# Autodesk Inventor assembly: intake_base_MIR
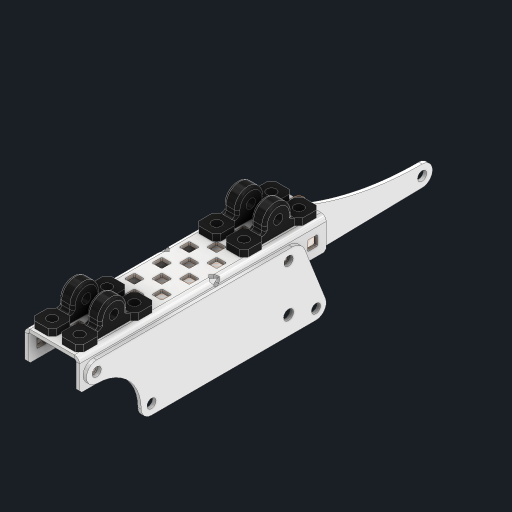
[picture p0: Inventor's stored thumbnail of the model, 512x512]
Saved by Autodesk Inventor 2024 (Build 280153000, 153)
## iProperties
Created: 2023-08-21
Part Number: intake_base_MIR
Document SubType Name: Assembly
Designer: Averey
Author: Averey
## Documents named in this file (5)
- D:\vex_robotics\hardware\cad\scrap_v0.1\intake\mirrored_parts\intake_base_MIR.iam
- D:\vex_robotics\hardware\cad\scrap_v0.1\intake\mirrored_parts\intake_base_MIR.ipt
- D:\vex_robotics\hardware\cad\scrap_v0.1\intake\mirrored_parts\intake_base_outer_MIR.ipt
- D:\vex_robotics\hardware\cad\scrap_v0.1\intake\mirrored_parts\LS Pillow Bearing Block_MIR.ipt
- D:\vex_robotics\hardware\cad\VEX-CAD-Inventor-1.41\Structure\C Channel\Aluminum 1x2x1\Alu C 1x2x1x9.ipt
## Components (7 placed, 4 different names)
1. intake_base_MIR:1 — Mate:7, Mate:8
2. intake_base_outer_MIR:1 — Insert:6, Mate:6
3. LS Pillow Bearing Block_MIR:1 — Insert:2, Mate:2
4. LS Pillow Bearing Block_MIR:2 — Insert:3, Mate:3
5. LS Pillow Bearing Block_MIR:3 — Insert:4, Mate:5
6. LS Pillow Bearing Block_MIR:4 — Insert:5, Mate:4
7. Alu C 1x2x1x9:1 — Insert:2, Mate:2, Insert:3, Mate:3, Insert:4, Insert:5, Mate:4, Mate:5, Insert:6, Mate:6, Mate:7, Mate:8
## Relationships (12: Mate 7, Insert 5)
- Insert:2: LS Pillow Bearing Block_MIR:1 ↔ Alu C 1x2x1x9:1
- Mate:2: LS Pillow Bearing Block_MIR:1 ↔ Alu C 1x2x1x9:1
- Insert:3: LS Pillow Bearing Block_MIR:2 ↔ Alu C 1x2x1x9:1
- Mate:3: LS Pillow Bearing Block_MIR:2 ↔ Alu C 1x2x1x9:1
- Insert:4: LS Pillow Bearing Block_MIR:3 ↔ Alu C 1x2x1x9:1
- Insert:5: LS Pillow Bearing Block_MIR:4 ↔ Alu C 1x2x1x9:1
- Mate:4: LS Pillow Bearing Block_MIR:4 ↔ Alu C 1x2x1x9:1
- Mate:5: LS Pillow Bearing Block_MIR:3 ↔ Alu C 1x2x1x9:1
- Insert:6: intake_base_outer_MIR:1 ↔ Alu C 1x2x1x9:1
- Mate:6: intake_base_outer_MIR:1 ↔ Alu C 1x2x1x9:1
- Mate:7: intake_base_MIR:1 ↔ Alu C 1x2x1x9:1
- Mate:8: intake_base_MIR:1 ↔ Alu C 1x2x1x9:1
